# Autodesk Inventor assembly: full
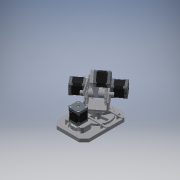
[picture p0: Inventor's stored thumbnail of the model, 180x180]
Saved by Autodesk Inventor 2019 (Build 230136000, 136)
## iProperties
Created: 2019-05-15
Part Number: full
Document SubType Name: Assembly
Designer: Nathan
Author: Nathan
## Documents named in this file (11)
- C:\Users\Nathan\workspace\fbd-brachium\cad\full.iam
- C:\Users\Nathan\workspace\fbd-brachium\cad\shoulder.ipt
- C:\Users\Nathan\workspace\fbd-brachium\cad\nema17.ipt
- C:\Users\Nathan\workspace\fbd-brachium\cad\base.ipt
- C:\Users\Nathan\workspace\fbd-brachium\cad\full\Design Accelerator\Spur Gears1.iam
- C:\Users\Nathan\workspace\fbd-brachium\cad\turntable_retention_shaft.ipt
- C:\Users\Nathan\workspace\fbd-brachium\cad\arm_proximal.ipt
- C:\Users\Nathan\workspace\fbd-brachium\cad\shoulder_gear_shaft.ipt
- C:\Users\Nathan\workspace\fbd-brachium\cad\arm_distal.ipt
- C:\Users\Nathan\workspace\fbd-brachium\cad\full\Design Accelerator\Spur Gears2.iam
- C:\Users\Nathan\workspace\fbd-brachium\cad\parameters.xlsx
## Components (13 placed, 8 different names)
1. shoulder:1 — Insert:1, Insert:2, Insert:3, Insert:4, Insert:5, Insert:8, Mate:4, Flush:1
2. nema17:1 — Insert:3, Insert:4
3. nema17:2 — Insert:1, Insert:2, Mate:5
4. base:1 — Insert:5, Insert:6, Insert:7, Mate:2, Mate:3
5. nema17:3 — Insert:6, Insert:7, Mate:1
6. Spur Gears:1 [sub-assembly] — Mate:1
7. turntable_retention_shaft:1 — Mate:3
8. turntable_retention_shaft:2 — Mate:2
9. arm_proximal:1 — Insert:8, Insert:9, Insert:10, Flush:2
10. nema17:4 — Insert:9, Insert:10, Insert:11
11. shoulder_gear_shaft:1 — Mate:4, Flush:1
12. arm_distal:1 — Insert:11
13. Spur Gears:2 [sub-assembly] — Mate:5, Flush:2
## Relationships (18: Insert 11, Mate 5, Flush 2)
- Insert:1: shoulder:1 ↔ nema17:2
- Insert:2: shoulder:1 ↔ nema17:2
- Insert:3: shoulder:1 ↔ nema17:1
- Insert:4: shoulder:1 ↔ nema17:1
- Insert:5: shoulder:1 ↔ base:1
- Insert:6: base:1 ↔ nema17:3
- Insert:7: base:1 ↔ nema17:3
- Mate:1: nema17:3 ↔ Spur Gears:1
- Mate:2: base:1 ↔ turntable_retention_shaft:2
- Mate:3: base:1 ↔ turntable_retention_shaft:1
- Insert:8: shoulder:1 ↔ arm_proximal:1
- Insert:9: arm_proximal:1 ↔ nema17:4
- Insert:10: arm_proximal:1 ↔ nema17:4
- Mate:4: shoulder:1 ↔ shoulder_gear_shaft:1
- Flush:1 (12.7 mm): shoulder:1 ↔ shoulder_gear_shaft:1
- Insert:11 (3.175 mm): nema17:4 ↔ arm_distal:1
- Mate:5: nema17:2 ↔ Spur Gears:2
- Flush:2: arm_proximal:1 ↔ Spur Gears:2
## Named parameters: base_length = 177.8 mm, base_width = 127 mm, base_height = 12.7 mm, base_cutout_contact_angle = 70 deg, base_cutout_diameter = 44.45 mm, turntable_motor_support_thickness = 3.175 mm, turntable_motor_support_width = 63.5 mm, turntable_motor_support_height = 19.05 mm, turntable_motor_boss = 25.4 mm, turntable_bed_depth = 3.175 mm, turntable_diameter = 101.6 mm, turntable_height = 9.525 mm, turntable_spurs = 6, turntable_spur_width = 6.35 mm, turntable_retention_shaft_diameter = 6.35 mm, turntable_retention_shaft_length = 152.4 mm, spine_diameter = 31.75 mm, spine_height = 25.4 mm, shoulder_length = 50.8 mm, shoulder_width = 69.85 mm, shoulder_wall_thickness = 4.7625 mm, shoulder_gear_diameter = 63.5 mm, shoulder_gear_thickness = 6.35 mm, shoulder_motor_gear_diameter = 25.4 mm, shoulder_gear_shaft_diameter = 12.7 mm, shoulder_motor_boss = 25.4 mm, arm_proximal_length = 203.2 mm, arm_proximal_thickness = 9.525 mm, arm_proximal_central_diameter = 25.4 mm, arm_proximal_motor_boss = 25.4 mm, arm_distal_length = 152.4 mm
